# Autodesk Inventor assembly: Ensamble Final Tensor Polea Dieku
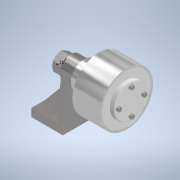
[picture p0: Inventor's stored thumbnail of the model, 180x180]
Saved by Autodesk Inventor 2021 (Build 250183000, 183)
## iProperties
Created: 2021-01-10
Part Number: Ensamble Final Tensor Polea Dieku
Document SubType Name: Assembly
Designer: dieku
Author: dieku
## Documents named in this file (3)
- C:\Users\dieku\Documents\GitHub\tallerDibujoIngenieria\Ensamble Final Tensor Polea Dieku.iam
- C:\Users\dieku\Documents\GitHub\tallerDibujoIngenieria\Ensambles\Cosa sin eje.iam
- C:\Users\dieku\Documents\GitHub\tallerDibujoIngenieria\Ensambles\Ensamble tensor + eje.iam
## Components (2 placed, 2 different names)
1. Cosa sin eje:1 [sub-assembly] — Insert:1
2. Ensamble tensor + eje:1 [sub-assembly] — Insert:1
## Relationships (1: Insert 1)
- Insert:1: Cosa sin eje:1 ↔ Ensamble tensor + eje:1
